# Autodesk Inventor assembly: Manilla
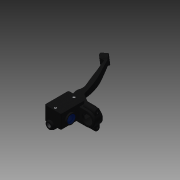
[picture p0: Inventor's stored thumbnail of the model, 180x180]
Saved by Autodesk Inventor 2016 (Build 200138000, 138)
## iProperties
Created: 2013-07-10
Part Number: Manilla
Document SubType Name: Assembly
Designer: Luis
Author: Luis
## Documents named in this file (10)
- C:\Users\Yann\Documents\GitHub\BIKAIR_CAD\Source\Front_Train\Brakes\Levers\Manilla.iam
- C:\Users\Yann\Documents\GitHub\BIKAIR_CAD\Source\Front_Train\Brakes\Levers\Base.ipt
- C:\Users\Yann\Documents\GitHub\BIKAIR_CAD\Source\Front_Train\Brakes\Levers\Goma.ipt
- C:\Users\Yann\Documents\GitHub\BIKAIR_CAD\Source\Front_Train\Brakes\Levers\Tapa.ipt
- C:\Users\Yann\Documents\GitHub\BIKAIR_CAD\Source\Front_Train\Brakes\Levers\MAN.ipt
- C:\Users\Yann\Documents\GitHub\BIKAIR_CAD\Source\Front_Train\Brakes\Levers\pIST.ipt
- C:\Users\Yann\Documents\GitHub\BIKAIR_CAD\Source\Front_Train\Brakes\Levers\Goma pist.ipt
- C:\Users\Yann\Documents\GitHub\BIKAIR_CAD\Source\Front_Train\Brakes\Levers\nivel.ipt
- C:\Users\Yann\Documents\GitHub\BIKAIR_CAD\Source\Front_Train\Brakes\Levers\Abrazadera.ipt
- C:\Users\Yann\Documents\GitHub\BIKAIR_CAD\Source\Front_Train\Brakes\Levers\Tornillo tapa.ipt
## Components (10 placed, 9 different names)
1. Base:1 — Insert:1, Insert:2, Insert:5, Insert:6, Insert:8, Insert:9, Insert:10
2. Goma:1 — Insert:1, Insert:2, Insert:3, Insert:4
3. Tapa:1 — Insert:3, Insert:4, Insert:11, Insert:12
4. MAN:1 — Insert:5, Tangent:1
5. pIST:1 — Insert:6, Insert:7, Tangent:1
6. Goma pist:1 — Insert:7
7. nivel:1 — Insert:8
8. Abrazadera:1 — Insert:9, Insert:10
9. Tornillo tapa:1 — Insert:11
10. Tornillo tapa:2 — Insert:12
## Relationships (13: Insert 12, Tangent 1)
- Insert:1: Base:1 ↔ Goma:1
- Insert:2: Base:1 ↔ Goma:1
- Insert:3: Goma:1 ↔ Tapa:1
- Insert:4: Goma:1 ↔ Tapa:1
- Insert:5: Base:1 ↔ MAN:1
- Insert:6: Base:1 ↔ pIST:1
- Insert:7: pIST:1 ↔ Goma pist:1
- Tangent:1: MAN:1 ↔ pIST:1
- Insert:8: Base:1 ↔ nivel:1
- Insert:9: Base:1 ↔ Abrazadera:1
- Insert:10: Base:1 ↔ Abrazadera:1
- Insert:11: Tapa:1 ↔ Tornillo tapa:1
- Insert:12: Tapa:1 ↔ Tornillo tapa:2
